# Autodesk Inventor assembly: Delta_Robot
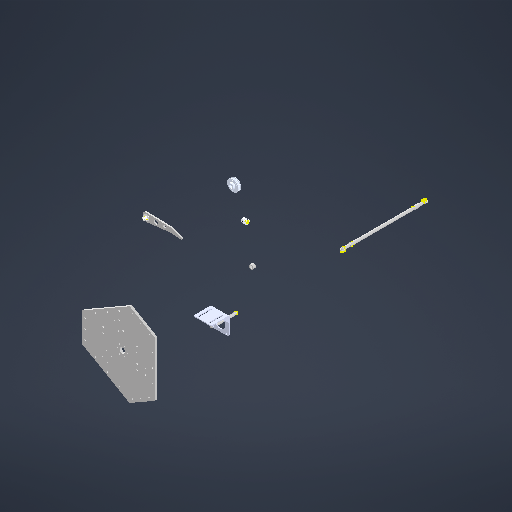
[picture p0: Inventor's stored thumbnail of the model, 512x512]
Saved by Autodesk Inventor 2027.1 (Build 311270010, 270A)
## iProperties
Created: 2026-08-09
Part Number: Delta_Robot
Document SubType Name: Assembly
Designer: MSI
Author: MSI
## Documents named in this file (14)
- C:\Users\MSI\Documents\MECHATRONICS\Tot_nghiep\Do_an_Delta.Robot_Dang_Rui_Bi\Thiết kế\Delta Part\Delta_Robot.iam
- C:\Users\MSI\Documents\MECHATRONICS\Tot_nghiep\Do_an_Delta.Robot_Dang_Rui_Bi\Thiết kế\Delta Part\khóa trục.ipt
- C:\Users\MSI\Documents\MECHATRONICS\Tot_nghiep\Do_an_Delta.Robot_Dang_Rui_Bi\Thiết kế\Delta Part\khớp nối.ipt
- C:\Users\MSI\Documents\MECHATRONICS\Tot_nghiep\Do_an_Delta.Robot_Dang_Rui_Bi\Thiết kế\Delta Part\Link1.ipt
- C:\Users\MSI\Documents\MECHATRONICS\Tot_nghiep\Do_an_Delta.Robot_Dang_Rui_Bi\Thiết kế\Delta Part\link2.ipt
- C:\Users\MSI\Documents\MECHATRONICS\Tot_nghiep\Do_an_Delta.Robot_Dang_Rui_Bi\Thiết kế\Delta Part\mặt bích.ipt
- C:\Users\MSI\Documents\MECHATRONICS\Tot_nghiep\Do_an_Delta.Robot_Dang_Rui_Bi\Thiết kế\Delta Part\trục đai.ipt
- C:\Users\MSI\Documents\MECHATRONICS\Tot_nghiep\Do_an_Delta.Robot_Dang_Rui_Bi\Thiết kế\Delta Part\chốt khớp nối.ipt
- C:\Users\MSI\Documents\MECHATRONICS\Tot_nghiep\Do_an_Delta.Robot_Dang_Rui_Bi\Thiết kế\Delta Part\đế gá step.ipt
- C:\Users\MSI\Documents\MECHATRONICS\Tot_nghiep\Do_an_Delta.Robot_Dang_Rui_Bi\Thiết kế\Delta Part\đế trên.ipt
- C:\Users\MSI\Documents\MECHATRONICS\Tot_nghiep\Do_an_Delta.Robot_Dang_Rui_Bi\Thiết kế\Delta Part\GT2_20T.ipt
- C:\Users\MSI\Documents\MECHATRONICS\Tot_nghiep\Do_an_Delta.Robot_Dang_Rui_Bi\Thiết kế\Delta Part\GT2_60.ipt
- C:\Users\MSI\Documents\MECHATRONICS\Tot_nghiep\Do_an_Delta.Robot_Dang_Rui_Bi\Thiết kế\Delta Part\khớp nối mắt trâu lỗ 4mm.iam
- C:\Users\MSI\Documents\Inventor\Content Center Files\R2027\en-US\IFI 513(2)\IFI 513 - M2.5x0.45 x 4(1) IA.ipt
## Components (19 placed, 13 different names)
1. khóa trục:1
2. Link1:1 — Mate:1, Mate:2, Mate:41, Mate:42, Mate:43, Mate:44, Mate:45, Insert:1, Insert:2, Insert:3, Insert:4
3. mặt bích:1 — Mate:1, Mate:2
4. trục đai:1
5. chốt khớp nối:1
6. đế gá step:1
7. đế trên:1
8. GT2_20T:1
9. GT2_60:1
10. khớp nối mắt trâu lỗ 4mm:11 [sub-assembly] — Mate:37, Mate:38
11. khớp nối mắt trâu lỗ 4mm:12 [sub-assembly] — Mate:39, Mate:40
12. link2:9
13. khớp nối:17 — Mate:39, Mate:40
14. khớp nối:18 — Mate:37, Mate:38
15. Cross Recessed Flat Countersunk Head Machine Screw - Type IA - Metric M2.5x0.45 x 4:1 — Mate:41, Insert:1
16. Cross Recessed Flat Countersunk Head Machine Screw - Type IA - Metric M2.5x0.45 x 4:2 — Mate:42
17. Cross Recessed Flat Countersunk Head Machine Screw - Type IA - Metric M2.5x0.45 x 4:3 — Mate:43, Insert:3
18. Cross Recessed Flat Countersunk Head Machine Screw - Type IA - Metric M2.5x0.45 x 4:4 — Mate:44, Insert:4
19. Cross Recessed Flat Countersunk Head Machine Screw - Type IA - Metric M2.5x0.45 x 4:5 — Mate:45, Insert:2
## Relationships (18: Mate 14, Insert 4)
- Mate:1: Link1:1 ↔ mặt bích:1
- Mate:2: Link1:1 ↔ mặt bích:1
- [Mate]: link2:9 ↔ khớp nối:18
- [Mate]: link2:9 ↔ khớp nối:17
- [Mate]: link2:9 ↔ khớp nối:17
- Mate:37: khớp nối mắt trâu lỗ 4mm:11 ↔ khớp nối:18
- Mate:38: khớp nối mắt trâu lỗ 4mm:11 ↔ khớp nối:18
- Mate:39: khớp nối mắt trâu lỗ 4mm:12 ↔ khớp nối:17
- Mate:40: khớp nối mắt trâu lỗ 4mm:12 ↔ khớp nối:17
- Mate:41: Link1:1 ↔ Cross Recessed Flat Countersunk Head Machine Screw - Type IA - Metric M2.5x0.45 x 4:1
- Mate:42: Link1:1 ↔ Cross Recessed Flat Countersunk Head Machine Screw - Type IA - Metric M2.5x0.45 x 4:2
- Mate:43: Link1:1 ↔ Cross Recessed Flat Countersunk Head Machine Screw - Type IA - Metric M2.5x0.45 x 4:3
- Mate:44: Link1:1 ↔ Cross Recessed Flat Countersunk Head Machine Screw - Type IA - Metric M2.5x0.45 x 4:4
- Mate:45: Link1:1 ↔ Cross Recessed Flat Countersunk Head Machine Screw - Type IA - Metric M2.5x0.45 x 4:5
- Insert:1: Link1:1 ↔ Cross Recessed Flat Countersunk Head Machine Screw - Type IA - Metric M2.5x0.45 x 4:1
- Insert:2: Link1:1 ↔ Cross Recessed Flat Countersunk Head Machine Screw - Type IA - Metric M2.5x0.45 x 4:5
- Insert:3: Link1:1 ↔ Cross Recessed Flat Countersunk Head Machine Screw - Type IA - Metric M2.5x0.45 x 4:3
- Insert:4: Link1:1 ↔ Cross Recessed Flat Countersunk Head Machine Screw - Type IA - Metric M2.5x0.45 x 4:4
## Named parameters: d24_d10 = 0 mm, d25_d12 = 0 mm, d26_d17 = 0 mm, Finish1_Area = 10.6896
note: some values were not read from the file. Shown as the stored number, unit unknown: "Finish1_Area".
